# Autodesk Inventor assembly: Robot4
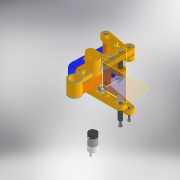
[picture p0: Inventor's stored thumbnail of the model, 180x180]
Saved by Autodesk Inventor 2021 (Build 250183000, 183)
## iProperties
Created: 2024-04-10
Part Number: Robot4
Document SubType Name: Assembly
Designer: Martin
Mass: 2207.07 g
Surface Area: 3653.09 cm^2
Volume: 938.659 cm^3
Density: 2.3513 g/cm^3
Author: Martin
## Documents named in this file (16)
- C:\Users\ASUS\OneDrive - Universidad de Antioquia\2024-1\Robótica\Proyecto\CAD\op1\Robot5.iam
- C:\Users\ASUS\OneDrive - Universidad de Antioquia\2024-1\Robótica\Proyecto\CAD\op1\BaseEnsamble.iam
- C:\Users\ASUS\OneDrive - Universidad de Antioquia\2024-1\Robótica\Proyecto\CAD\op1\EslabonCodoTrasero.ipt
- C:\Users\ASUS\OneDrive - Universidad de Antioquia\2024-1\Robótica\Proyecto\CAD\op1\EslabonRodillaCadera.ipt
- C:\Users\ASUS\OneDrive - Universidad de Antioquia\2024-1\Robótica\Proyecto\CAD\op1\EslabonRuedaRodilla.ipt
- C:\Users\ASUS\OneDrive - Universidad de Antioquia\2024-1\Robótica\Proyecto\CAD\37d-gearmotor-19-30-encoder.ipt
- C:\Users\ASUS\OneDrive - Universidad de Antioquia\2024-1\Robótica\Proyecto\CAD\Resorte.ipt
- C:\Users\ASUS\Documents\Inventor\Content Center Files\R2021\en-US\GB_T 276-94 60000-RS and LS\Bearing 61900-LS GB_T 276-94.ipt
- C:\Users\ASUS\Documents\Inventor\Content Center Files\R2021\en-US\AS 1111\AS 1111 - M8 x 90.ipt
- C:\Users\ASUS\Documents\Inventor\Content Center Files\R2021\en-US\ISO 1207(2)\ISO 1207 - M8 x 50.ipt
- C:\Users\ASUS\Documents\Inventor\Content Center Files\R2021\en-US\AS 1112 (2)\AS 1112 - M8  Type 5.ipt
- C:\Users\ASUS\OneDrive - Universidad de Antioquia\2024-1\Robótica\Proyecto\CAD\op1\EslabonCodoTrasero_MIR3.ipt
- C:\Users\ASUS\OneDrive - Universidad de Antioquia\2024-1\Robótica\Proyecto\CAD\op1\EslabonRodillaCadera_MIR3.ipt
- C:\Users\ASUS\OneDrive - Universidad de Antioquia\2024-1\Robótica\Proyecto\CAD\op1\EslabonRuedaRodilla_MIR3.ipt
- C:\Users\ASUS\OneDrive - Universidad de Antioquia\2024-1\Robótica\Proyecto\CAD\37d-gearmotor-19-30-encoder_MIR3.ipt
- C:\Users\ASUS\OneDrive - Universidad de Antioquia\2024-1\Robótica\Proyecto\CAD\Resorte_MIR4.ipt
## Components (37 placed, 15 different names)
1. BaseEnsamble:1 [sub-assembly] — Mate:11, Mate:12, Mate:13, Insert:1
2. EslabonCodoTrasero:1 — Mate:9, Mate:10, Mate:13, Mate:22, Mate:23, Mate:28, Mate:29, Insert:2, Insert:3
3. EslabonRodillaCadera:1 — Mate:6, Mate:7, Mate:11, Mate:12, Mate:14, Mate:15
4. EslabonRuedaRodilla:1 — Mate:3, Mate:4, Mate:6, Mate:7, Mate:8, Mate:9, Mate:10, Mate:16, Mate:17, Mate:18, Mate:19, Mate:20, Mate:21, Mate:24, Mate:25, Mate:26, Mate:27, Mate:61, Mate:62
5. 37d-gearmotor-19-30-encoder:1 — Mate:3, Mate:4
6. Resorte:1 — Mate:8
7. Rolling bearing GB/T 276-1994 Type 60000-RS and LS 61900-LS:1 — Mate:14, Mate:15
8. Rolling bearing GB/T 276-1994 Type 60000-RS and LS 61900-LS:2 — Mate:18, Mate:19
9. Rolling bearing GB/T 276-1994 Type 60000-RS and LS 61900-LS:3 — Mate:22, Mate:23, Mate:31
10. Rolling bearing GB/T 276-1994 Type 60000-RS and LS 61900-LS:4 — Mate:16, Mate:17
11. Rolling bearing GB/T 276-1994 Type 60000-RS and LS 61900-LS:5 — Mate:20, Mate:21
12. AS 1111 - Metric M8 x 90:1 — Mate:24, Mate:25, Mate:32
13. ISO 1207 M8 x 50:1 — Mate:26, Mate:27, Mate:30
14. AS 1111 - Metric M8 x 90:2 — Mate:28, Mate:29
15. AS 1112 (2) - Metric M8  Type 5:1 — Insert:1
16. AS 1112 (2) - Metric M8  Type 5:2 — Mate:30, Mate:31
17. AS 1112 (2) - Metric M8  Type 5:3 — Insert:2
18. AS 1112 (2) - Metric M8  Type 5:4 — Insert:3
19. AS 1112 (2) - Metric M8  Type 5:5 — Mate:32
20. EslabonCodoTrasero_MIR3:1 — Mate:65, Mate:66, Mate:76, Mate:77, Mate:86, Mate:87, Insert:4, Insert:5
21. EslabonRodillaCadera_MIR3:1 — Mate:67, Mate:68, Mate:72, Mate:73
22. EslabonRuedaRodilla_MIR3:1 — Mate:63, Mate:64, Mate:65, Mate:66, Mate:67, Mate:68, Mate:69, Mate:70, Mate:71, Mate:74, Mate:75, Mate:78, Mate:79, Mate:80, Mate:81, Mate:82, Mate:83, Mate:84, Mate:85
23. 37d-gearmotor-19-30-encoder_MIR3:1 — Mate:69, Mate:70
24. Resorte_MIR4:1 — Mate:71
25. Rolling bearing GB/T 276-1994 Type 60000-RS and LS 61900-LS:6 — Mate:72, Mate:73
26. Rolling bearing GB/T 276-1994 Type 60000-RS and LS 61900-LS:7 — Mate:74, Mate:75
27. Rolling bearing GB/T 276-1994 Type 60000-RS and LS 61900-LS:8 — Mate:76, Mate:77, Mate:88
28. Rolling bearing GB/T 276-1994 Type 60000-RS and LS 61900-LS:9 — Mate:78, Mate:79
29. Rolling bearing GB/T 276-1994 Type 60000-RS and LS 61900-LS:10 — Mate:80, Mate:81
30. AS 1111 - Metric M8 x 90:3 — Mate:82, Mate:83, Mate:90
31. ISO 1207 M8 x 50:2 — Mate:84, Mate:85, Mate:89
32. AS 1111 - Metric M8 x 90:4 — Mate:86, Mate:87
33. AS 1112 (2) - Metric M8  Type 5:6
34. AS 1112 (2) - Metric M8  Type 5:7 — Mate:88, Mate:89
35. AS 1112 (2) - Metric M8  Type 5:8 — Insert:4
36. AS 1112 (2) - Metric M8  Type 5:9 — Insert:5
37. AS 1112 (2) - Metric M8  Type 5:10 — Mate:90
## Relationships (64: Mate 59, Insert 5)
- Mate:3: EslabonRuedaRodilla:1 ↔ 37d-gearmotor-19-30-encoder:1
- Mate:4: EslabonRuedaRodilla:1 ↔ 37d-gearmotor-19-30-encoder:1
- Mate:6: EslabonRodillaCadera:1 ↔ EslabonRuedaRodilla:1
- Mate:7 (46 mm): EslabonRodillaCadera:1 ↔ EslabonRuedaRodilla:1
- Mate:8: EslabonRuedaRodilla:1 ↔ Resorte:1
- Mate:9: EslabonCodoTrasero:1 ↔ EslabonRuedaRodilla:1
- Mate:10 (10 mm): EslabonCodoTrasero:1 ↔ EslabonRuedaRodilla:1
- Mate:11: BaseEnsamble:1 ↔ EslabonRodillaCadera:1
- Mate:12 (1 mm): BaseEnsamble:1 ↔ EslabonRodillaCadera:1
- Mate:13: BaseEnsamble:1 ↔ EslabonCodoTrasero:1
- Mate:14: EslabonRodillaCadera:1 ↔ Rolling bearing GB/T 276-1994 Type 60000-RS and LS 61900-LS:1
- Mate:15: EslabonRodillaCadera:1 ↔ Rolling bearing GB/T 276-1994 Type 60000-RS and LS 61900-LS:1
- Mate:16: EslabonRuedaRodilla:1 ↔ Rolling bearing GB/T 276-1994 Type 60000-RS and LS 61900-LS:4
- Mate:17: EslabonRuedaRodilla:1 ↔ Rolling bearing GB/T 276-1994 Type 60000-RS and LS 61900-LS:4
- Mate:18: EslabonRuedaRodilla:1 ↔ Rolling bearing GB/T 276-1994 Type 60000-RS and LS 61900-LS:2
- Mate:19: EslabonRuedaRodilla:1 ↔ Rolling bearing GB/T 276-1994 Type 60000-RS and LS 61900-LS:2
- Mate:20: EslabonRuedaRodilla:1 ↔ Rolling bearing GB/T 276-1994 Type 60000-RS and LS 61900-LS:5
- Mate:21: EslabonRuedaRodilla:1 ↔ Rolling bearing GB/T 276-1994 Type 60000-RS and LS 61900-LS:5
- Mate:22: EslabonCodoTrasero:1 ↔ Rolling bearing GB/T 276-1994 Type 60000-RS and LS 61900-LS:3
- Mate:23: EslabonCodoTrasero:1 ↔ Rolling bearing GB/T 276-1994 Type 60000-RS and LS 61900-LS:3
- Mate:24: EslabonRuedaRodilla:1 ↔ AS 1111 - Metric M8 x 90:1
- Mate:25: EslabonRuedaRodilla:1 ↔ AS 1111 - Metric M8 x 90:1
- Mate:26: EslabonRuedaRodilla:1 ↔ ISO 1207 M8 x 50:1
- Mate:27: EslabonRuedaRodilla:1 ↔ ISO 1207 M8 x 50:1
- Mate:28: EslabonCodoTrasero:1 ↔ AS 1111 - Metric M8 x 90:2
- Mate:29: EslabonCodoTrasero:1 ↔ AS 1111 - Metric M8 x 90:2
- Insert:1: BaseEnsamble:1 ↔ AS 1112 (2) - Metric M8  Type 5:1
- Mate:30: ISO 1207 M8 x 50:1 ↔ AS 1112 (2) - Metric M8  Type 5:2
- Mate:31: Rolling bearing GB/T 276-1994 Type 60000-RS and LS 61900-LS:3 ↔ AS 1112 (2) - Metric M8  Type 5:2
- Insert:2: EslabonCodoTrasero:1 ↔ AS 1112 (2) - Metric M8  Type 5:3
- Insert:3: EslabonCodoTrasero:1 ↔ AS 1112 (2) - Metric M8  Type 5:4
- Mate:32: AS 1111 - Metric M8 x 90:1 ↔ AS 1112 (2) - Metric M8  Type 5:5
- Mate:61: EslabonRuedaRodilla:1
- Mate:62 (-9 mm): EslabonRuedaRodilla:1
- Mate:63 (-9 mm): EslabonRuedaRodilla_MIR3:1
- Mate:64: EslabonRuedaRodilla_MIR3:1
- Mate:65 (10 mm): EslabonCodoTrasero_MIR3:1 ↔ EslabonRuedaRodilla_MIR3:1
- Mate:66: EslabonCodoTrasero_MIR3:1 ↔ EslabonRuedaRodilla_MIR3:1
- Mate:67 (46 mm): EslabonRodillaCadera_MIR3:1 ↔ EslabonRuedaRodilla_MIR3:1
- Mate:68: EslabonRodillaCadera_MIR3:1 ↔ EslabonRuedaRodilla_MIR3:1
- Mate:69: EslabonRuedaRodilla_MIR3:1 ↔ 37d-gearmotor-19-30-encoder_MIR3:1
- Mate:70: EslabonRuedaRodilla_MIR3:1 ↔ 37d-gearmotor-19-30-encoder_MIR3:1
- Mate:71: EslabonRuedaRodilla_MIR3:1 ↔ Resorte_MIR4:1
- Mate:72: EslabonRodillaCadera_MIR3:1 ↔ Rolling bearing GB/T 276-1994 Type 60000-RS and LS 61900-LS:6
- Mate:73: EslabonRodillaCadera_MIR3:1 ↔ Rolling bearing GB/T 276-1994 Type 60000-RS and LS 61900-LS:6
- Mate:74: EslabonRuedaRodilla_MIR3:1 ↔ Rolling bearing GB/T 276-1994 Type 60000-RS and LS 61900-LS:7
- Mate:75: EslabonRuedaRodilla_MIR3:1 ↔ Rolling bearing GB/T 276-1994 Type 60000-RS and LS 61900-LS:7
- Mate:76: EslabonCodoTrasero_MIR3:1 ↔ Rolling bearing GB/T 276-1994 Type 60000-RS and LS 61900-LS:8
- Mate:77: EslabonCodoTrasero_MIR3:1 ↔ Rolling bearing GB/T 276-1994 Type 60000-RS and LS 61900-LS:8
- Mate:78: EslabonRuedaRodilla_MIR3:1 ↔ Rolling bearing GB/T 276-1994 Type 60000-RS and LS 61900-LS:9
- Mate:79: EslabonRuedaRodilla_MIR3:1 ↔ Rolling bearing GB/T 276-1994 Type 60000-RS and LS 61900-LS:9
- Mate:80: EslabonRuedaRodilla_MIR3:1 ↔ Rolling bearing GB/T 276-1994 Type 60000-RS and LS 61900-LS:10
- Mate:81: EslabonRuedaRodilla_MIR3:1 ↔ Rolling bearing GB/T 276-1994 Type 60000-RS and LS 61900-LS:10
- Mate:82: EslabonRuedaRodilla_MIR3:1 ↔ AS 1111 - Metric M8 x 90:3
- Mate:83: EslabonRuedaRodilla_MIR3:1 ↔ AS 1111 - Metric M8 x 90:3
- Mate:84: EslabonRuedaRodilla_MIR3:1 ↔ ISO 1207 M8 x 50:2
- Mate:85: EslabonRuedaRodilla_MIR3:1 ↔ ISO 1207 M8 x 50:2
- Mate:86: EslabonCodoTrasero_MIR3:1 ↔ AS 1111 - Metric M8 x 90:4
- Mate:87: EslabonCodoTrasero_MIR3:1 ↔ AS 1111 - Metric M8 x 90:4
- Mate:88: Rolling bearing GB/T 276-1994 Type 60000-RS and LS 61900-LS:8 ↔ AS 1112 (2) - Metric M8  Type 5:7
- Mate:89: ISO 1207 M8 x 50:2 ↔ AS 1112 (2) - Metric M8  Type 5:7
- Insert:4: EslabonCodoTrasero_MIR3:1 ↔ AS 1112 (2) - Metric M8  Type 5:8
- Insert:5: EslabonCodoTrasero_MIR3:1 ↔ AS 1112 (2) - Metric M8  Type 5:9
- Mate:90: AS 1111 - Metric M8 x 90:3 ↔ AS 1112 (2) - Metric M8  Type 5:10
